# Autodesk Inventor assembly: Bearing_Holder
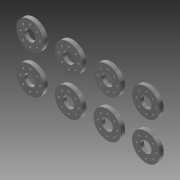
[picture p0: Inventor's stored thumbnail of the model, 180x180]
Saved by Autodesk Inventor 2013 (Build 170138000, 138)
## iProperties
Created: 2014-04-21
Part Number: Bearing_Holder
Document SubType Name: Assembly
Designer: andou
Author: andou
## Documents named in this file (2)
- C:\Users\andou\Documents\GitHub\Robotics-Project\design\RoboticsProject\project_4\cnc_data\Bearing_Holder_8.iam
- C:\Users\andou\Documents\GitHub\Robotics-Project\design\RoboticsProject\project_4\cnc_data\Leg_Bearing_Holder.ipt
## Components (8 placed, 1 different names)
1. Leg_Bearing_Holder:16
2. Leg_Bearing_Holder:17
3. Leg_Bearing_Holder:18
4. Leg_Bearing_Holder:19
5. Leg_Bearing_Holder:20
6. Leg_Bearing_Holder:21
7. Leg_Bearing_Holder:22
8. Leg_Bearing_Holder:23
## Component patterns: (8 elements, first: Leg_Bearing_Holder:16)
